# Autodesk Inventor assembly: LigthtCart-assembly
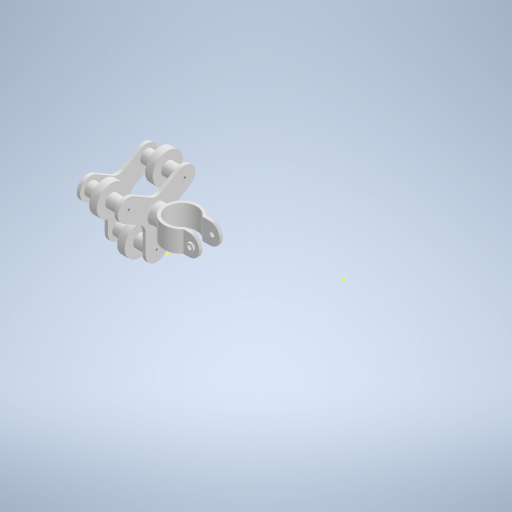
[picture p0: Inventor's stored thumbnail of the model, 512x512]
Saved by Autodesk Inventor 2023 (Build 270158000, 158)
## iProperties
Created: 2023-05-02
Part Number: LigthtCart-assembly
Document SubType Name: Assembly
Designer: ringl
Author: ringl
## Documents named in this file (4)
- C:\Users\ringl\Documents\Uni Classes\Y3S2\EE318-Project\EE318-Project\CAD\LightCart\LigthtCart-assembly.iam
- C:\Users\ringl\Documents\Uni Classes\Y3S2\EE318-Project\EE318-Project\CAD\LightCart\Grabber(changed).ipt
- C:\Users\ringl\Documents\Uni Classes\Y3S2\EE318-Project\EE318-Project\CAD\LightCart\triangle connection (changed).ipt
- C:\Users\ringl\Documents\Uni Classes\Y3S2\EE318-Project\EE318-Project\CAD\LightCart\bearing-test.ipt
## Components (5 placed, 3 different names)
1. Grabber(changed):1 — Mate:1, Mate:2
2. triangle connection (changed):1 — Mate:1, Mate:2, Mate:3, Mate:4, Mate:5, Mate:6, Mate:7, Mate:8
3. bearing-test:1 — Mate:3, Mate:6
4. bearing-test:2 — Mate:4, Mate:7
5. bearing-test:3 — Mate:5, Mate:8
## Relationships (8: Mate 8)
- Mate:1: Grabber(changed):1 ↔ triangle connection (changed):1
- Mate:2: Grabber(changed):1 ↔ triangle connection (changed):1
- Mate:3: triangle connection (changed):1 ↔ bearing-test:1
- Mate:4: triangle connection (changed):1 ↔ bearing-test:2
- Mate:5: triangle connection (changed):1 ↔ bearing-test:3
- Mate:6 (12.5 mm): triangle connection (changed):1 ↔ bearing-test:1
- Mate:7 (12.5 mm): triangle connection (changed):1 ↔ bearing-test:2
- Mate:8 (12.5 mm): triangle connection (changed):1 ↔ bearing-test:3
